# Autodesk Inventor assembly: PlanetaryAssembly
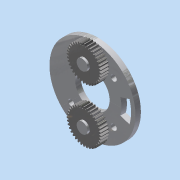
[picture p0: Inventor's stored thumbnail of the model, 180x180]
Saved by Autodesk Inventor 2015 (Build 190159000, 159)
## iProperties
Created: 2015-12-24
Part Number: PlanetaryAssembly
Document SubType Name: Assembly
Designer: Raphael
Author: Raphael
## Documents named in this file (3)
- \\psf\Home\Documents\electric-skateboard\CAD\HubMotor\PlanetaryAssembly.iam
- \\psf\Home\Documents\electric-skateboard\CAD\HubMotor\PlanetaryCarrier.ipt
- \\psf\Home\Documents\electric-skateboard\CAD\HubMotor\PlanetGear.ipt
## Components (3 placed, 2 different names)
1. PlanetaryCarrier:1 — Mate:1, Mate:2, Mate:3, Mate:4
2. PlanetGear:1 — Mate:1, Mate:3
3. PlanetGear:2 — Mate:2, Mate:4
## Relationships (4: Mate 4)
- Mate:1: PlanetaryCarrier:1 ↔ PlanetGear:1
- Mate:2: PlanetaryCarrier:1 ↔ PlanetGear:2
- Mate:3 (0.254 mm): PlanetaryCarrier:1 ↔ PlanetGear:1
- Mate:4 (0.254 mm): PlanetaryCarrier:1 ↔ PlanetGear:2
